# Autodesk Inventor assembly: mb_mother_board
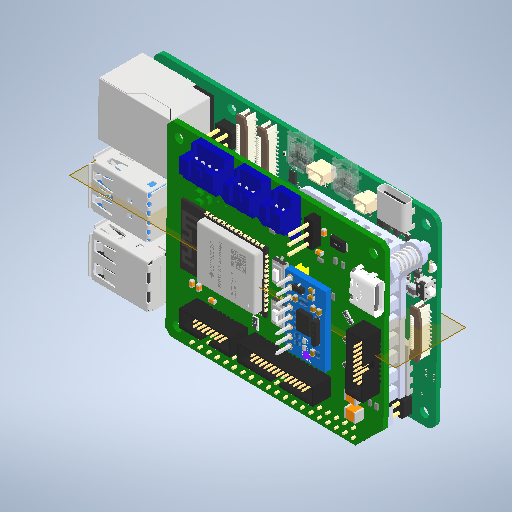
[picture p0: Inventor's stored thumbnail of the model, 512x512]
Saved by Autodesk Inventor 2025 (Build 290162000, 162)
## iProperties
Created: 2026-07-21
Part Number: mb_mother_board
Document SubType Name: Assembly
Designer: garin
Author: garin
## Documents named in this file (4)
- C:\Users\garin\Documents\Git\TheseusV2_Maze\Construction\Theseus_v2\mother_board\mb_mother_board.iam
- C:\Users\garin\Documents\Git\TheseusV2_Maze\Construction\Theseus_v2\mother_board\rpi-5b_no_graphics.ipt
- C:\Users\garin\Documents\Git\TheseusV2_Maze\Construction\Theseus_v2\mother_board\Heatsink+fan RPi-5.ipt
- C:\Users\garin\Documents\Git\TheseusV2_Maze\Schematic\TSE_mother_board\model\TSE_mother_board_final.iam
## Components (3 placed, 3 different names)
1. rpi-5b_no_graphics:1 — Совмещение:1, Совмещение:2, Угол:1, Совмещение:52, Совмещение:53, Совмещение:54
2. Heatsink+fan RPi-5:1 — Совмещение:1, Совмещение:2, Угол:1
3. TSE_mother_board_final:1 [sub-assembly] — Совмещение:52, Совмещение:53, Совмещение:54
## Relationships (6: Mate 5, Angle 1)
- Совмещение:1 [Mate]: rpi-5b_no_graphics:1 ↔ Heatsink+fan RPi-5:1
- Совмещение:2 [Mate]: rpi-5b_no_graphics:1 ↔ Heatsink+fan RPi-5:1
- Угол:1 [Angle] (0 deg): rpi-5b_no_graphics:1 ↔ Heatsink+fan RPi-5:1
- Совмещение:52 [Mate] (3 mm): rpi-5b_no_graphics:1 ↔ TSE_mother_board_final:1
- Совмещение:53 [Mate]: rpi-5b_no_graphics:1 ↔ TSE_mother_board_final:1
- Совмещение:54 [Mate]: rpi-5b_no_graphics:1 ↔ TSE_mother_board_final:1
